# Autodesk Inventor assembly: TW1
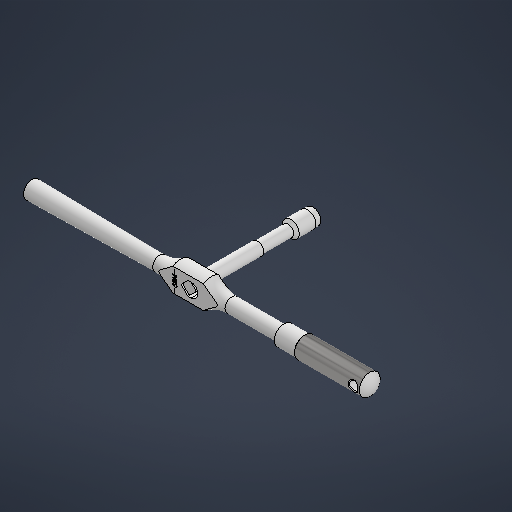
[picture p0: Inventor's stored thumbnail of the model, 512x512]
Saved by Autodesk Inventor 2025.3 (Build 293356000, 356)
## iProperties
Created: 2025-05-04
Part Number: TW1
Document SubType Name: Assembly
Designer: fablabadmin
Description: Tap wrench
Stock Number: -
Author: Benjamin Solar
Title: WEDU
Revision Number: 1
## Documents named in this file (6)
- C:\Users\fablabadmin\Documents\_Benjamin_S\_3dCAD\HHVerkstad\TapWrench1\TW1.iam
- C:\Users\fablabadmin\Documents\_Benjamin_S\_3dCAD\HHVerkstad\TapWrench1\TW1-001.ipt
- C:\Users\fablabadmin\Documents\_Benjamin_S\_3dCAD\HHVerkstad\TapWrench1\TW1-002.ipt
- C:\Users\fablabadmin\Documents\_Benjamin_S\_3dCAD\HHVerkstad\TapWrench1\TW1-003.ipt
- C:\Users\fablabadmin\Documents\_Benjamin_S\_3dCAD\HHVerkstad\TapWrench1\TW1-004.ipt
- C:\Users\fablabadmin\Documents\_Benjamin_S\_3dCAD\HHVerkstad\TapWrench1\E002M12.ipt
## Components (5 placed, 5 different names)
1. TW1-001:1 — Mate:1, Angle:1, Mate:3, Mate:4, Mate:5, Mate:6, Mate:7
2. TW1-002:1 — Mate:1, Angle:1, Mate:2, Tangent:1, Mate:8
3. TW1-003:1 — Mate:2, Mate:3
4. TW1-004:1 — Mate:4, Angle:2, Tangent:1
5. E002M12:1 — Mate:5, Mate:6, Mate:7, Mate:8
## Relationships (11: Mate 8, Angle 2, Tangent 1)
- Mate:1: TW1-001:1 ↔ TW1-002:1
- Angle:1 (0 deg): TW1-001:1 ↔ TW1-002:1
- Mate:2: TW1-002:1 ↔ TW1-003:1
- Mate:3: TW1-001:1 ↔ TW1-003:1
- Mate:4: TW1-001:1 ↔ TW1-004:1
- Angle:2 (0 deg): TW1-004:1
- Tangent:1: TW1-002:1 ↔ TW1-004:1
- Mate:5: TW1-001:1 ↔ E002M12:1
- Mate:6: TW1-001:1 ↔ E002M12:1
- Mate:7: TW1-001:1 ↔ E002M12:1
- Mate:8: TW1-002:1 ↔ E002M12:1
